# Autodesk Inventor assembly: ADSK-MH-10049
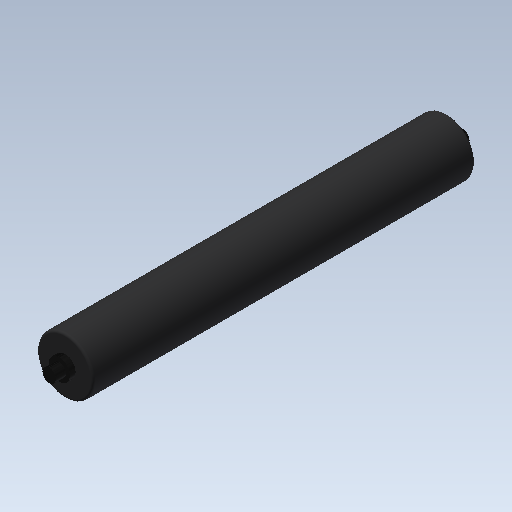
[picture p0: Inventor's stored thumbnail of the model, 512x512]
Saved by Autodesk Inventor 2020.2 (Build 242310000, 310)
## iProperties
Created: 2008-03-29
Part Number: ADSK-MH-10049
Document SubType Name: Assembly
Designer: R.O'Mahony
Description: Transfer Roller
Engineer: Demir Ali
Checked By: Demir Ali
Company: Autodesk Ltd
Author: R.O'Mahony
Keywords: Roller Conveyor
Revision Number: A
## Documents named in this file (3)
- C:\Users\peter\source\repos\InventorDA-FLC\Dataset\Discharge Conveyor\ADSK-MH-10049.iam
- C:\Users\peter\source\repos\InventorDA-FLC\Dataset\Discharge Conveyor\ADSK-MH-10049.ipt
- C:\Users\peter\source\repos\InventorDA-FLC\Dataset\Discharge Conveyor\ADSK-MH-10044.ipt
## Components (2 placed, 2 different names)
1. Transfer Roller — Mate:1, Mate:2
2. Transfer Roller Shaft — Mate:1, Mate:2
## Relationships (2: Mate 2)
- Mate:1: Transfer Roller ↔ Transfer Roller Shaft
- Mate:2: Transfer Roller ↔ Transfer Roller Shaft
